# Autodesk Inventor assembly: CameraAndLightRingMount
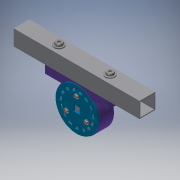
[picture p0: Inventor's stored thumbnail of the model, 180x180]
Saved by Autodesk Inventor 2019.3 (Build 233278000, 278)
## iProperties
Created: 2018-12-21
Part Number: CameraAndLightRingMount
Document SubType Name: Assembly
Designer: steele
Author: steele
## Documents named in this file (15)
- C:\git\CAD-Development\robSteele\ShapeWays\FRC\PiCameraAndLightRingMount\CameraAndLightRingMount.iam
- c:\git\CAD-MfgResources\ThingiVerse\Raspberry_Pi_Camera_Module_v2.1_Model\files\RPi_Camera_Module_v2.iam
- C:\git\CAD-Development\robSteele\ShapeWays\FRC\PiCameraAndLightRingMount\MountForLightRingAndPiCamera.ipt
- C:\git\CAD-Development\robSteele\ShapeWays\FRC\PiCameraAndLightRingMount\MountCover.ipt
- C:\git\CAD-Development\robSteele\ShapeWays\FRC\PiCameraAndLightRingMount\RaspberryPiCameraModel.ipt
- C:\git\CAD-Development\robSteele\ShapeWays\FRC\PiCameraAndLightRingMount\AlumBracket1x1.ipt
- C:\git\CAD-Development\robSteele\ShapeWays\FRC\PiCameraAndLightRingMount\AndyMarkLightRing2018.ipt
- C:\git\CAD-Development\robSteele\ShapeWays\FRC\PiCameraAndLightRingMount\7712K620_BATTERY HOLDER.ipt
- c:\git\CAD-MfgResources\McMaster-Carr\BrassHeatSetInsertForPlastic\2-56 94459A240_BRASS HEAT-SET INSERT FOR PLASTIC.ipt
- C:\git\CAD-Development\robSteele\ShapeWays\FRC\PiCameraAndLightRingMount\CameraAndLightRingMount\Design Accelerator\Bolted Connection5.iam
- c:\git\CAD-MfgResources\McMaster-Carr\BrassHeatSetInsertForPlastic\6-32 94459A290_BRASS HEAT-SET INSERT FOR PLASTIC.ipt
- C:\git\CAD-Development\robSteele\ShapeWays\FRC\PiCameraAndLightRingMount\CameraAndLightRingMount\Design Accelerator\Bolted Connection7.iam
- C:\git\CAD-Development\robSteele\ShapeWays\FRC\PiCameraAndLightRingMount\CameraAndLightRingMount\Design Accelerator\Bolted Connection8.iam
- c:\git\CAD-MfgResources\McMaster-Carr\BrassHeatSetInsertForPlastic\1_4-20 0_312 94459A370_BRASS HEAT-SET INSERT FOR PLASTIC.ipt
- C:\git\CAD-Development\robSteele\ShapeWays\FRC\PiCameraAndLightRingMount\CameraAndLightRingMount\Design Accelerator\Bolted Connection9.iam
## Components (22 placed, 11 different names)
1. RPi_Camera_Module_v2:1 [sub-assembly] — Mate:1, Mate:2, Mate:3
2. MountForLightRingAndPiCamera:1 — Mate:1, Mate:2, Mate:3, Mate:4, Mate:7, Mate:8, Mate:9, Mate:13, Insert:3, Flush:1, Mate:16, Insert:4, Flush:2, Mate:23, Flush:3, Mate:24, Insert:5, Insert:6, Insert:7, Insert:8, Insert:9, Insert:10, Insert:11, Insert:12, Insert:13, Insert:14, Insert:15
3. MountCover:1 — Mate:4, Mate:13, Insert:3, Mate:27, Mate:28
4. RaspberryPiCameraModel:1 — Mate:7, Mate:8, Mate:9, Mate:25, Mate:26
5. AlumBracket1x1:1 — Flush:1, Mate:16, Flush:2, Mate:31
6. AndyMarkLightRing2018:1 — Insert:4
7. 7712K620_BATTERY HOLDER:1 — Mate:23, Flush:3, Mate:24, Mate:29, Mate:30
8. 2-56 94459A240_BRASS HEAT-SET INSERT FOR PLASTIC:1 — Insert:5
9. 2-56 94459A240_BRASS HEAT-SET INSERT FOR PLASTIC:2 — Insert:6
10. 2-56 94459A240_BRASS HEAT-SET INSERT FOR PLASTIC:3 — Insert:8
11. 2-56 94459A240_BRASS HEAT-SET INSERT FOR PLASTIC:4 — Insert:7
12. Bolted Connection:1 [sub-assembly] — Mate:25, Mate:26
13. 6-32 94459A290_BRASS HEAT-SET INSERT FOR PLASTIC:1 — Insert:9
14. 6-32 94459A290_BRASS HEAT-SET INSERT FOR PLASTIC:2 — Insert:10
15. 6-32 94459A290_BRASS HEAT-SET INSERT FOR PLASTIC:3 — Insert:11
16. 6-32 94459A290_BRASS HEAT-SET INSERT FOR PLASTIC:4 — Insert:13
17. 6-32 94459A290_BRASS HEAT-SET INSERT FOR PLASTIC:5 — Insert:12
18. Bolted Connection:2 [sub-assembly] — Mate:27, Mate:28
19. Bolted Connection:3 [sub-assembly] — Mate:29, Mate:30
20. 1_4-20 0_312 94459A370_BRASS HEAT-SET INSERT FOR PLASTIC:1 — Insert:15
21. 1_4-20 0_312 94459A370_BRASS HEAT-SET INSERT FOR PLASTIC:2 — Insert:14, Mate:32
22. Bolted Connection:4 [sub-assembly] — Mate:31, Mate:32
## Relationships (35: Mate 19, Insert 13, Flush 3)
- Mate:1: RPi_Camera_Module_v2:1 ↔ MountForLightRingAndPiCamera:1
- Mate:2 (1 mm): RPi_Camera_Module_v2:1 ↔ MountForLightRingAndPiCamera:1
- Mate:3 (1 mm): RPi_Camera_Module_v2:1 ↔ MountForLightRingAndPiCamera:1
- Mate:4: MountForLightRingAndPiCamera:1 ↔ MountCover:1
- Mate:7 (1 mm): MountForLightRingAndPiCamera:1 ↔ RaspberryPiCameraModel:1
- Mate:8 (1 mm): MountForLightRingAndPiCamera:1 ↔ RaspberryPiCameraModel:1
- Mate:9: MountForLightRingAndPiCamera:1 ↔ RaspberryPiCameraModel:1
- Mate:13: MountForLightRingAndPiCamera:1 ↔ MountCover:1
- Insert:3: MountForLightRingAndPiCamera:1 ↔ MountCover:1
- Flush:1: MountForLightRingAndPiCamera:1 ↔ AlumBracket1x1:1
- Mate:16: MountForLightRingAndPiCamera:1 ↔ AlumBracket1x1:1
- Insert:4: MountForLightRingAndPiCamera:1 ↔ AndyMarkLightRing2018:1
- Flush:2: MountForLightRingAndPiCamera:1 ↔ AlumBracket1x1:1
- Mate:23: MountForLightRingAndPiCamera:1 ↔ 7712K620_BATTERY HOLDER:1
- Flush:3: MountForLightRingAndPiCamera:1 ↔ 7712K620_BATTERY HOLDER:1
- Mate:24 (-2.1463 mm): MountForLightRingAndPiCamera:1 ↔ 7712K620_BATTERY HOLDER:1
- Insert:5: MountForLightRingAndPiCamera:1 ↔ 2-56 94459A240_BRASS HEAT-SET INSERT FOR PLASTIC:1
- Insert:6: MountForLightRingAndPiCamera:1 ↔ 2-56 94459A240_BRASS HEAT-SET INSERT FOR PLASTIC:2
- Insert:7: MountForLightRingAndPiCamera:1 ↔ 2-56 94459A240_BRASS HEAT-SET INSERT FOR PLASTIC:4
- Insert:8: MountForLightRingAndPiCamera:1 ↔ 2-56 94459A240_BRASS HEAT-SET INSERT FOR PLASTIC:3
- Mate:25: RaspberryPiCameraModel:1 ↔ Bolted Connection:1
- Mate:26: RaspberryPiCameraModel:1 ↔ Bolted Connection:1
- Insert:9: MountForLightRingAndPiCamera:1 ↔ 6-32 94459A290_BRASS HEAT-SET INSERT FOR PLASTIC:1
- Insert:10: MountForLightRingAndPiCamera:1 ↔ 6-32 94459A290_BRASS HEAT-SET INSERT FOR PLASTIC:2
- Insert:11: MountForLightRingAndPiCamera:1 ↔ 6-32 94459A290_BRASS HEAT-SET INSERT FOR PLASTIC:3
- Insert:12: MountForLightRingAndPiCamera:1 ↔ 6-32 94459A290_BRASS HEAT-SET INSERT FOR PLASTIC:5
- Insert:13: MountForLightRingAndPiCamera:1 ↔ 6-32 94459A290_BRASS HEAT-SET INSERT FOR PLASTIC:4
- Mate:27: MountCover:1 ↔ Bolted Connection:2
- Mate:28: MountCover:1 ↔ Bolted Connection:2
- Mate:29: 7712K620_BATTERY HOLDER:1 ↔ Bolted Connection:3
- Mate:30: 7712K620_BATTERY HOLDER:1 ↔ Bolted Connection:3
- Insert:14: MountForLightRingAndPiCamera:1 ↔ 1_4-20 0_312 94459A370_BRASS HEAT-SET INSERT FOR PLASTIC:2
- Insert:15: MountForLightRingAndPiCamera:1 ↔ 1_4-20 0_312 94459A370_BRASS HEAT-SET INSERT FOR PLASTIC:1
- Mate:31: AlumBracket1x1:1 ↔ Bolted Connection:4
- Mate:32: 1_4-20 0_312 94459A370_BRASS HEAT-SET INSERT FOR PLASTIC:2 ↔ Bolted Connection:4
## Named parameters: LightRingExternalDiameter = 60 mm, LightRingInternalDiameter = 44 mm, LightRingDepth = 1.2 mm, LightRingSpacing = 2 mm, MountExternalDiameter = 70 mm, LightRingCenterRadius = 26 mm, CameraCenterToTop = 9.462 mm, CameraCenterToBottom = 14.4 mm, CameraCenterToSide = 12.5 mm, CameraLensToSurface = 5 mm, CameraBoardThickness = 1 mm, CameraRibbonHolderThickness = 2.4 mm, LightRingWireDiameter = 8 mm, CameraHoleDiameter = 2.2 mm, CameraSpacing = 1 mm
